# Autodesk Inventor assembly: 00_X02598_LEGOmini_CityGuy
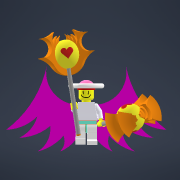
[picture p0: Inventor's stored thumbnail of the model, 180x180]
Saved by Autodesk Inventor 2022 (Build 260153000, 153)
## iProperties
Created: 2022-02-05
Part Number: 00_X02598_LEGOmini_CityGuy
Document SubType Name: Assembly
Designer: Jason
Author: Jason
## Documents named in this file (6)
- D:\D-disk\pomelo\大一\下學期\機械設計製圖\110033226_LEGOmini\110033226_LEGOmini_天使\110033226_LEGOmini_天使.iam
- D:\D-disk\pomelo\大一\下學期\機械設計製圖\110033226_LEGOmini\110033226_LEGOmini_天使\110033226_LEGOmini_天使下半身.iam
- D:\D-disk\pomelo\大一\下學期\機械設計製圖\110033226_LEGOmini\110033226_LEGOmini_天使\110033226_LEGOmini_天使上半身.iam
- D:\D-disk\pomelo\大一\下學期\機械設計製圖\110033226_LEGOmini\110033226_LEGOmini_天使\110033226_LEGOmini_天使頭.ipt
- D:\D-disk\pomelo\大一\下學期\機械設計製圖\110033226_LEGOmini\110033226_LEGOmini_天使\110033226_LEGOmini_光環.ipt
- D:\D-disk\pomelo\大一\下學期\機械設計製圖\110033226_LEGOmini\110033226_LEGOmini_天使\110033226_LEGOmini_天使權杖.ipt
## Components (6 placed, 5 different names)
1. 110033226_LEGOmini_天使下半身:1 [sub-assembly] — 貼合:1, 齊平:1, 齊平:2
2. 110033226_LEGOmini_天使上半身:1 [sub-assembly] — 貼合:1, 齊平:1, 齊平:2, 插入:1, 貼合:2, 貼合:3
3. 110033226_LEGOmini_天使頭:1 — 插入:1, 插入:2
4. 110033226_LEGOmini_光環:1 — 插入:2
5. 110033226_LEGOmini_天使權杖:1 — 貼合:2
6. 110033226_LEGOmini_天使權杖:2 — 貼合:3
## Relationships (7: Mate 3, Flush 2, Insert 2)
- 貼合:1 [Mate]: 110033226_LEGOmini_天使下半身:1 ↔ 110033226_LEGOmini_天使上半身:1
- 齊平:1 [Flush]: 110033226_LEGOmini_天使下半身:1 ↔ 110033226_LEGOmini_天使上半身:1
- 齊平:2 [Flush]: 110033226_LEGOmini_天使下半身:1 ↔ 110033226_LEGOmini_天使上半身:1
- 插入:1 [Insert]: 110033226_LEGOmini_天使上半身:1 ↔ 110033226_LEGOmini_天使頭:1
- 插入:2 [Insert]: 110033226_LEGOmini_天使頭:1 ↔ 110033226_LEGOmini_光環:1
- 貼合:2 [Mate]: 110033226_LEGOmini_天使上半身:1 ↔ 110033226_LEGOmini_天使權杖:1
- 貼合:3 [Mate]: 110033226_LEGOmini_天使上半身:1 ↔ 110033226_LEGOmini_天使權杖:2
